# Autodesk Inventor assembly: Complete_Assembly
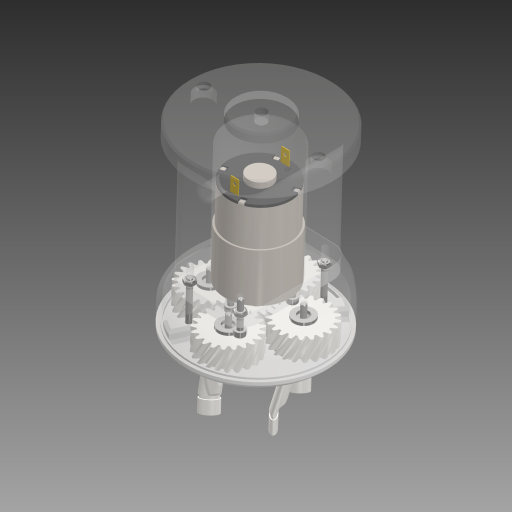
[picture p0: Inventor's stored thumbnail of the model, 512x512]
Saved by Autodesk Inventor 2024 (Build 280153000, 153)
## iProperties
Created: 2024-03-16
Part Number: Complete_Assembly
Document SubType Name: Assembly
Designer: Faber
Author: Faber
## Documents named in this file (14)
- C:\Users\Bluex\Documents\GitHub\Autonome_Robotter\3D_inventor_robor_hånd\Complete_Assembly.iam
- C:\Users\Bluex\Documents\GitHub\Autonome_Robotter\3D_inventor_robor_hånd\Motor_Enclosure.ipt
- C:\Users\Bluex\Documents\GitHub\Autonome_Robotter\3D_inventor_robor_hånd\Content Center Files\ISO 4032 - M3DIN EN.ipt
- C:\Users\Bluex\Documents\GitHub\Autonome_Robotter\3D_inventor_robor_hånd\Motor-HG37-300-AB-00\3D\HG37-300-AB-00\HG37-300-AB-00.iam
- C:\Users\Bluex\Documents\GitHub\Autonome_Robotter\3D_inventor_robor_hånd\Gear_Enclosure.ipt
- C:\Users\Bluex\Documents\GitHub\Autonome_Robotter\3D_inventor_robor_hånd\Content Center Files\DIN EN ISO 4762 - M3 x 8.ipt
- C:\Users\Bluex\Documents\Inventor\Content Center Files\R2024\en-US\DIN 125-1  A\DIN 125 - A 6,4.ipt
- C:\Users\Bluex\Documents\GitHub\Autonome_Robotter\3D_inventor_robor_hånd\Gear_Assembly\Design Accelerator\Spur Gear21.ipt
- C:\Users\Bluex\Documents\Inventor\Content Center Files\R2024\en-US\DIN 125-1  A\DIN 125 - A 4,3.ipt
- C:\Users\Bluex\Documents\Inventor\Content Center Files\R2024\en-US\ISO 4762(1)\DIN EN ISO 4762 - M3 x 20.ipt
- C:\Users\Bluex\Documents\GitHub\Autonome_Robotter\3D_inventor_robor_hånd\Content Center Files\DIN EN ISO 4762 - M3 x 16.ipt
- C:\Users\Bluex\Documents\GitHub\Autonome_Robotter\3D_inventor_robor_hånd\Gear_Enclosure_Lid.ipt
- C:\Users\Bluex\Documents\GitHub\Autonome_Robotter\3D_inventor_robor_hånd\Gear_Assembly\Design Accelerator\Spur Gear11.ipt
- C:\Users\Bluex\Documents\GitHub\Autonome_Robotter\3D_inventor_robor_hånd\Content Center Files\DIN EN ISO 4762 - M3 x 25.ipt
## Components (32 placed, 13 different names)
1. Motor_Enclosure:1 — Mate:1, Mate:2, Mate:3, Mate:4, Mate:5, Mate:6, Mate:7, Mate:8, Mate:9, Flush:1, Mate:11, Mate:12, Mate:13, Angle:1, Angle:2
2. DIN EN 24032 M3:1 — Mate:1, Mate:2
3. DIN EN 24032 M3:2 — Mate:7, Mate:8
4. DIN EN 24032 M3:3 — Mate:5, Mate:6
5. DIN EN 24032 M3:4 — Mate:3, Mate:4
6. HG37-300-AB-00:1 [sub-assembly] — Mate:9, Flush:1, Mate:10, Mate:14, Insert:20
7. Gear_Enclosure:1 — Mate:10, Mate:11, Mate:12, Mate:14, Insert:1, Mate:15, Mate:16, Mate:17, Insert:2, Insert:3, Insert:4, Insert:9, Insert:18, Insert:19, Mate:18, Mate:19, Mate:20
8. DIN EN ISO 4762 M3 x 16:1 — Insert:19
9. DIN EN ISO 4762 M3 x 16:2 — Insert:18
10. DIN EN ISO 4762 M3 x 8:1 — Insert:1
11. DIN EN ISO 4762 M3 x 8:2 — Mate:16
12. DIN EN ISO 4762 M3 x 8:3 — Mate:15
13. DIN 125-1 A A 6,4:1 — Mate:17, Insert:6, Insert:9
14. DIN 125-1 A A 6,4:2 — Insert:2, Insert:5
15. DIN 125-1 A A 6,4:3 — Insert:4, Insert:7
16. DIN 125-1 A A 6,4:4 — Insert:3, Insert:8
17. Spur Gear1:1 — Insert:20, Rotation:1, Rotation:3, Rotation:4, Rotation:5
18. Spur Gear2:1 — Insert:5, Insert:11, Rotation:1
19. Spur Gear2:2 — Insert:6, Insert:10, Rotation:4
20. Spur Gear2:3 — Insert:7, Insert:12, Rotation:3
21. Spur Gear2:4 — Insert:8, Insert:13, Rotation:5
22. DIN 125-1 A A 4,3:1 — Insert:10, Insert:14
23. DIN 125-1 A A 4,3:2 — Insert:13, Insert:16
24. DIN 125-1 A A 4,3:3 — Insert:12, Insert:15
25. DIN 125-1 A A 4,3:4 — Insert:11, Insert:17
26. DIN EN ISO 4762 M3 x 20:1 — Insert:16
27. DIN EN ISO 4762 M3 x 20:2 — Insert:17
28. DIN EN ISO 4762 M3 x 20:3 — Insert:15
29. DIN EN ISO 4762 M3 x 20:4 — Insert:14
30. Gear_Enclosure_Lid:1 — Mate:18, Mate:19, Mate:20, Insert:21, Insert:22
31. DIN EN ISO 4762 M3 x 25:1 — Insert:21
32. DIN EN ISO 4762 M3 x 25:2 — Insert:22
## Relationships (49: Insert 22, Mate 20, RelateRotation 4, Angle 2, Flush 1)
- Mate:1: Motor_Enclosure:1 ↔ DIN EN 24032 M3:1
- Mate:2: Motor_Enclosure:1 ↔ DIN EN 24032 M3:1
- Mate:3: Motor_Enclosure:1 ↔ DIN EN 24032 M3:4
- Mate:4: Motor_Enclosure:1 ↔ DIN EN 24032 M3:4
- Mate:5: Motor_Enclosure:1 ↔ DIN EN 24032 M3:3
- Mate:6: Motor_Enclosure:1 ↔ DIN EN 24032 M3:3
- Mate:7: Motor_Enclosure:1 ↔ DIN EN 24032 M3:2
- Mate:8: Motor_Enclosure:1 ↔ DIN EN 24032 M3:2
- Mate:9: Motor_Enclosure:1 ↔ HG37-300-AB-00:1
- Flush:1: Motor_Enclosure:1 ↔ HG37-300-AB-00:1
- Mate:10: HG37-300-AB-00:1 ↔ Gear_Enclosure:1
- Mate:11: Motor_Enclosure:1 ↔ Gear_Enclosure:1
- Mate:12: Motor_Enclosure:1 ↔ Gear_Enclosure:1
- Mate:13: Motor_Enclosure:1
- Angle:1 (1.76 deg): Motor_Enclosure:1
- Mate:14: HG37-300-AB-00:1 ↔ Gear_Enclosure:1
- Angle:2 (0 deg): Motor_Enclosure:1
- Insert:1: Gear_Enclosure:1 ↔ DIN EN ISO 4762 M3 x 8:1
- Mate:15: Gear_Enclosure:1 ↔ DIN EN ISO 4762 M3 x 8:3
- Mate:16: Gear_Enclosure:1 ↔ DIN EN ISO 4762 M3 x 8:2
- Mate:17: Gear_Enclosure:1 ↔ DIN 125-1 A A 6,4:1
- Insert:2: Gear_Enclosure:1 ↔ DIN 125-1 A A 6,4:2
- Insert:3: Gear_Enclosure:1 ↔ DIN 125-1 A A 6,4:4
- Insert:4: Gear_Enclosure:1 ↔ DIN 125-1 A A 6,4:3
- Insert:5: DIN 125-1 A A 6,4:2 ↔ Spur Gear2:1
- Insert:6: DIN 125-1 A A 6,4:1 ↔ Spur Gear2:2
- Insert:7: DIN 125-1 A A 6,4:3 ↔ Spur Gear2:3
- Insert:8: DIN 125-1 A A 6,4:4 ↔ Spur Gear2:4
- Insert:9: Gear_Enclosure:1 ↔ DIN 125-1 A A 6,4:1
- Insert:10: Spur Gear2:2 ↔ DIN 125-1 A A 4,3:1
- Insert:11: Spur Gear2:1 ↔ DIN 125-1 A A 4,3:4
- Insert:12: Spur Gear2:3 ↔ DIN 125-1 A A 4,3:3
- Insert:13: Spur Gear2:4 ↔ DIN 125-1 A A 4,3:2
- Insert:14: DIN 125-1 A A 4,3:1 ↔ DIN EN ISO 4762 M3 x 20:4
- Insert:15: DIN 125-1 A A 4,3:3 ↔ DIN EN ISO 4762 M3 x 20:3
- Insert:16: DIN 125-1 A A 4,3:2 ↔ DIN EN ISO 4762 M3 x 20:1
- Insert:17: DIN 125-1 A A 4,3:4 ↔ DIN EN ISO 4762 M3 x 20:2
- Insert:18: Gear_Enclosure:1 ↔ DIN EN ISO 4762 M3 x 16:2
- Insert:19: Gear_Enclosure:1 ↔ DIN EN ISO 4762 M3 x 16:1
- Mate:18: Gear_Enclosure:1 ↔ Gear_Enclosure_Lid:1
- Mate:19: Gear_Enclosure:1 ↔ Gear_Enclosure_Lid:1
- Mate:20: Gear_Enclosure:1 ↔ Gear_Enclosure_Lid:1
- Insert:20 (1 mm): HG37-300-AB-00:1 ↔ Spur Gear1:1
- Rotation:1 [RelateRotation] (0.5714 ul): Spur Gear1:1 ↔ Spur Gear2:1
- Rotation:3 [RelateRotation] (0.5714 ul): Spur Gear1:1 ↔ Spur Gear2:3
- Rotation:4 [RelateRotation] (0.5714 ul): Spur Gear1:1 ↔ Spur Gear2:2
- Rotation:5 [RelateRotation] (0.5714 ul): Spur Gear1:1 ↔ Spur Gear2:4
- Insert:21: Gear_Enclosure_Lid:1 ↔ DIN EN ISO 4762 M3 x 25:1
- Insert:22: Gear_Enclosure_Lid:1 ↔ DIN EN ISO 4762 M3 x 25:2
